# Autodesk Inventor assembly: Exentric strap
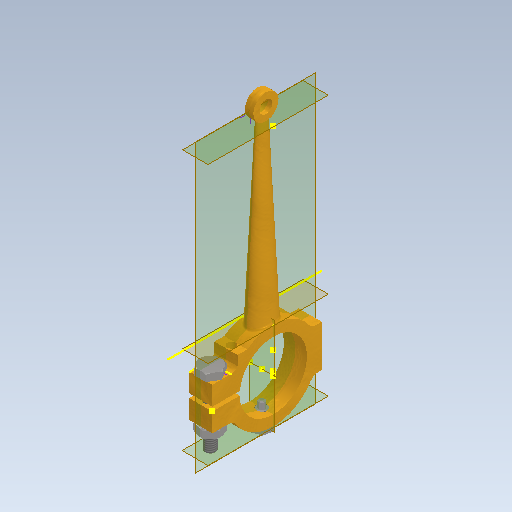
[picture p0: Inventor's stored thumbnail of the model, 512x512]
Saved by Autodesk Inventor 2020 (Build 240168000, 168)
## iProperties
Created: 2021-10-27
Part Number: Exentric strap
Document SubType Name: Assembly
Designer: simon.erikssonwestl
Author: simon.erikssonwestl
## Documents named in this file (5)
- C:\Users\simon.erikssonwestl\Documents\Inventor\Ång\Assemblies\Exentric strap.iam
- C:\Users\simon.erikssonwestl\Documents\Inventor\Ång\Part19.ipt
- C:\Users\simon.erikssonwestl\Documents\Inventor\Content Center Files\R2020\en-US\AS 1110\AS 1110 - M2,5 x 16.ipt
- C:\Users\simon.erikssonwestl\Documents\Inventor\Content Center Files\R2020\en-US\AS 1112 (2)\AS 1112 - M2,5  Type 5.ipt
- C:\Users\simon.erikssonwestl\Documents\Inventor\Ång\Part20.ipt
## Components (4 placed, 4 different names)
1. Part19:1 — Mate:1, Mate:2, Mate:4, Mate:5, Mate:6
2. AS 1110 - Metric M2,5 x 16:1 — Mate:1, Mate:2, Mate:3
3. AS 1112 (2) - Metric M2,5  Type 5:1 — Mate:3, Mate:4
4. Part20:1 — Mate:5, Mate:6
## Relationships (6: Mate 6)
- Mate:1: Part19:1 ↔ AS 1110 - Metric M2,5 x 16:1
- Mate:2: Part19:1 ↔ AS 1110 - Metric M2,5 x 16:1
- Mate:3: AS 1110 - Metric M2,5 x 16:1 ↔ AS 1112 (2) - Metric M2,5  Type 5:1
- Mate:4: Part19:1 ↔ AS 1112 (2) - Metric M2,5  Type 5:1
- Mate:5: Part19:1 ↔ Part20:1
- Mate:6 (10.5 mm): Part19:1 ↔ Part20:1
